# Autodesk Inventor assembly: Kitai
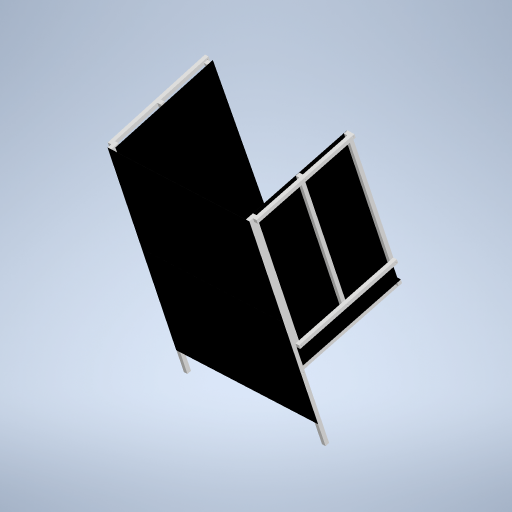
[picture p0: Inventor's stored thumbnail of the model, 512x512]
Saved by Autodesk Inventor 2023 (Build 270158000, 158)
## iProperties
Created: 2022-10-15
Part Number: Kitai
Document SubType Name: Assembly
Designer: banru
Author: banru
## Documents named in this file (9)
- C:\Users\banru\Documents\workspace\Contactless\Inventor\Kitai.iam
- C:\Users\banru\Documents\workspace\Contactless\Inventor\Dai.ipt
- C:\Users\banru\Documents\workspace\Contactless\Inventor\Yoko.ipt
- C:\Users\banru\Documents\workspace\Contactless\Inventor\Tate.ipt
- C:\Users\banru\Documents\workspace\Contactless\Inventor\Ita.ipt
- C:\Users\banru\Documents\workspace\Contactless\Inventor\YokoUe.ipt
- C:\Users\banru\Documents\workspace\Contactless\Inventor\SokuYoko.ipt
- C:\Users\banru\Documents\workspace\Contactless\Inventor\SokuTate.ipt
- C:\Users\banru\Documents\workspace\Contactless\Inventor\SokuYokoUe.ipt
## Components (21 placed, 8 different names)
1. Dai:1 — 挿入:2, 挿入:3, 挿入:11, 挿入:14
2. Dai:2 — メイト:7, メイト:8, フラッシュ:16, 挿入:1, 挿入:8, メイト:11, フラッシュ:17, 挿入:12, 挿入:13
3. Yoko:1 — 挿入:1, 挿入:2, メイト:10
4. Tate:1 — 挿入:3, 挿入:10
5. Ita:1 — メイト:12, フラッシュ:18, フラッシュ:19
6. Ita:2 — メイト:7, メイト:9, メイト:11, フラッシュ:17
7. Ita:4 — メイト:8, メイト:9, フラッシュ:16
8. YokoUe:1 — 挿入:9, 挿入:10, メイト:12, フラッシュ:18, フラッシュ:19
9. SokuYoko:1 — 挿入:11, 挿入:14, 挿入:17, 挿入:18, フラッシュ:20
10. SokuYoko:2 — 挿入:12, 挿入:13, 挿入:15, 挿入:16, フラッシュ:21
11. SokuTate:1 — 挿入:15, 挿入:20, フラッシュ:21, 挿入:25
12. SokuTate:2 — 挿入:16, 挿入:21, 挿入:22
13. SokuTate:3 — 挿入:18, メイト:13, 挿入:23, フラッシュ:22
14. SokuTate:4 — 挿入:17, 挿入:19, フラッシュ:20, 挿入:24
15. SokuYokoUe:1 — 挿入:19, メイト:13, メイト:14, フラッシュ:23
16. SokuYokoUe:2 — 挿入:20, 挿入:21, メイト:15, フラッシュ:24, フラッシュ:25
17. SokuYokoUe:3 — 挿入:23, 挿入:24
18. SokuYokoUe:4 — 挿入:22, 挿入:25
19. Ita:5 — メイト:14, フラッシュ:22, フラッシュ:23
20. Ita:6 — メイト:15, フラッシュ:24, フラッシュ:25
21. Tate:2 — 挿入:8, メイト:10, 挿入:9
## Relationships (40: Insert 21, Flush 10, Mate 9)
- メイト:7 [Mate]: Dai:2 ↔ Ita:2
- メイト:8 [Mate]: Dai:2 ↔ Ita:4
- メイト:9 [Mate]: Ita:2 ↔ Ita:4
- フラッシュ:16 [Flush]: Dai:2 ↔ Ita:4
- 挿入:1 [Insert]: Dai:2 ↔ Yoko:1
- 挿入:2 [Insert]: Dai:1 ↔ Yoko:1
- 挿入:3 [Insert]: Dai:1 ↔ Tate:1
- 挿入:8 [Insert]: Dai:2 ↔ Tate:2
- メイト:10 [Mate]: Yoko:1 ↔ Tate:2
- 挿入:9 [Insert]: YokoUe:1 ↔ Tate:2
- 挿入:10 [Insert]: Tate:1 ↔ YokoUe:1
- メイト:11 [Mate]: Dai:2 ↔ Ita:2
- フラッシュ:17 [Flush]: Dai:2 ↔ Ita:2
- メイト:12 [Mate]: Ita:1 ↔ YokoUe:1
- フラッシュ:18 [Flush]: Ita:1 ↔ YokoUe:1
- フラッシュ:19 [Flush]: Ita:1 ↔ YokoUe:1
- 挿入:11 [Insert]: Dai:1 ↔ SokuYoko:1
- 挿入:12 [Insert]: Dai:2 ↔ SokuYoko:2
- 挿入:13 [Insert]: Dai:2 ↔ SokuYoko:2
- 挿入:14 [Insert]: Dai:1 ↔ SokuYoko:1
- 挿入:15 [Insert]: SokuYoko:2 ↔ SokuTate:1
- 挿入:16 [Insert]: SokuYoko:2 ↔ SokuTate:2
- 挿入:17 [Insert]: SokuYoko:1 ↔ SokuTate:4
- 挿入:18 [Insert]: SokuYoko:1 ↔ SokuTate:3
- 挿入:19 [Insert]: SokuTate:4 ↔ SokuYokoUe:1
- 挿入:20 [Insert]: SokuTate:1 ↔ SokuYokoUe:2
- メイト:13 [Mate]: SokuTate:3 ↔ SokuYokoUe:1
- 挿入:21 [Insert]: SokuTate:2 ↔ SokuYokoUe:2
- 挿入:22 [Insert]: SokuTate:2 ↔ SokuYokoUe:4
- 挿入:23 [Insert]: SokuTate:3 ↔ SokuYokoUe:3
- フラッシュ:20 [Flush]: SokuYoko:1 ↔ SokuTate:4
- フラッシュ:21 [Flush]: SokuYoko:2 ↔ SokuTate:1
- 挿入:24 [Insert]: SokuTate:4 ↔ SokuYokoUe:3
- 挿入:25 [Insert]: SokuTate:1 ↔ SokuYokoUe:4
- メイト:14 [Mate]: SokuYokoUe:1 ↔ Ita:5
- フラッシュ:22 [Flush]: SokuTate:3 ↔ Ita:5
- フラッシュ:23 [Flush]: SokuYokoUe:1 ↔ Ita:5
- メイト:15 [Mate]: SokuYokoUe:2 ↔ Ita:6
- フラッシュ:24 [Flush]: SokuYokoUe:2 ↔ Ita:6
- フラッシュ:25 [Flush]: SokuYokoUe:2 ↔ Ita:6
